# Autodesk Inventor assembly: 組合
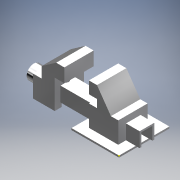
[picture p0: Inventor's stored thumbnail of the model, 180x180]
Saved by Autodesk Inventor 2017 (Build 210142000, 142)
## iProperties
Part Number: 組合
Material: 一般
Document SubType Name: Assembly
Designer: user
Author: user
## Documents named in this file (6)
- D:\410571040\組合.iam
- D:\410571040\完成\ㄇ形件.ipt
- D:\410571040\完成\小虎鉗-右側.ipt
- D:\410571040\完成\小虎鉗-左側.ipt
- D:\410571040\完成\底板.ipt
- D:\410571040\完成\螺桿.ipt
## Components (5 placed, 5 different names)
1. ㄇ形件:1 — 剛性:1, 剛性:2
2. 小虎鉗-右側:1 — 剛性:2, 圓柱:1
3. 小虎鉗-左側:1 — 旋轉:1, 剛性:1
4. 底板:1 — 旋轉:1
5. 螺桿:1 — 圓柱:1
## Relationships (4: WeldJoint 2, RevoluteJoint 1, CylindricalJoint 1)
- 旋轉:1 [RevoluteJoint]: 小虎鉗-左側:1 ↔ 底板:1
- 剛性:1 [WeldJoint]: ㄇ形件:1 ↔ 小虎鉗-左側:1
- 剛性:2 [WeldJoint]: ㄇ形件:1 ↔ 小虎鉗-右側:1
- 圓柱:1 [CylindricalJoint]: 小虎鉗-右側:1 ↔ 螺桿:1
